# Autodesk Inventor assembly: still pipe
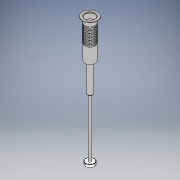
[picture p0: Inventor's stored thumbnail of the model, 180x180]
Saved by Autodesk Inventor 2018 (Build 220112000, 112)
## iProperties
Created: 2019-01-14
Part Number: still pipe
Document SubType Name: Assembly
Designer: Admin
Author: Admin
## Documents named in this file (5)
- C:\Users\Admin\Documents\Cryostat\CAD\still pipe.iam
- C:\Users\Admin\Documents\Cryostat\CAD\KF50 bellows.ipt
- C:\Users\Admin\Documents\Cryostat\CAD\still pipe small.iam.ipt
- C:\Users\Admin\Documents\Cryostat\CAD\universal connector.ipt
- still pipe small.iam
## Components (3 placed, 3 different names)
1. KF50 bellows:1 — Mate:1
2. still pipe small.iam:1 — Mate:1, Mate:2, Flush:1
3. universal connector:1 — Mate:2, Flush:1
## Relationships (3: Mate 2, Flush 1)
- Mate:1: KF50 bellows:1 ↔ still pipe small.iam:1
- Mate:2: still pipe small.iam:1 ↔ universal connector:1
- Flush:1: still pipe small.iam:1 ↔ universal connector:1
